# Autodesk Inventor assembly: gantry_frame
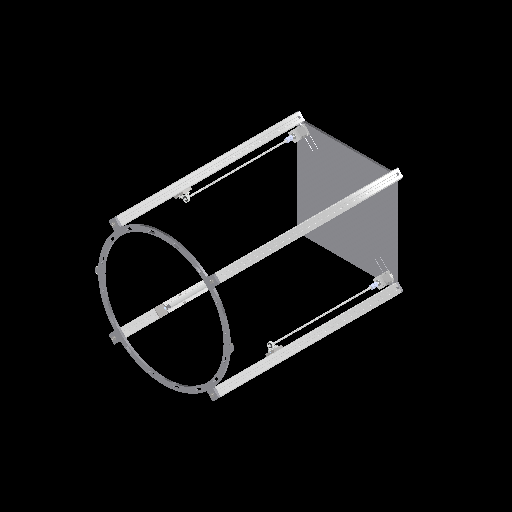
[picture p0: Inventor's stored thumbnail of the model, 512x512]
Saved by Autodesk Inventor 2026.1 (Build 301233000, 233)
## iProperties
Created: 2025-09-18
Part Number: gantry_frame
Document SubType Name: Assembly
Designer: drago
Author: drago
## Documents named in this file (11)
- C:\Users\drago\Desktop\_QIST4500_Multidisciplinary_Team_Project\Proteox MX magnet positioner CAD\magnet_positioner_cad_design\gantry_frame\gantry_frame.iam
- C:\Users\drago\Desktop\_QIST4500_Multidisciplinary_Team_Project\Proteox MX magnet positioner CAD\magnet_positioner_cad_design\gantry_frame\square_bar.ipt
- C:\Users\drago\Desktop\_QIST4500_Multidisciplinary_Team_Project\Proteox MX magnet positioner CAD\magnet_positioner_cad_design\gantry_frame\base_plate.ipt
- C:\Users\drago\Desktop\_QIST4500_Multidisciplinary_Team_Project\Proteox MX magnet positioner CAD\magnet_positioner_cad_design\z_rail\z_rail.iam
- C:\Users\drago\Desktop\_QIST4500_Multidisciplinary_Team_Project\Proteox MX magnet positioner CAD\magnet_positioner_cad_design\gantry_frame\full_ring.iam
- C:\Users\drago\Desktop\_QIST4500_Multidisciplinary_Team_Project\Proteox MX magnet positioner CAD\magnet_positioner_cad_design\z_translator\z_translator.iam
- C:\Users\drago\Documents\Inventor\Content Center Files\R2026\en-US\ISO 7089\ISO 7089 - 8 - 140 HV(1).ipt
- C:\Users\drago\Documents\Inventor\Content Center Files\R2026\en-US\ISO 4762(2)\ISO 4762 - M8 x 30ISO.ipt
- C:\Users\drago\Documents\Inventor\Content Center Files\R2026\en-US\ISO 7089\ISO 7089 - 3 - 140 HV(1).ipt
- C:\Users\drago\Documents\Inventor\Content Center Files\R2026\en-US\ISO 4762(2)\ISO 4762 - M3 x 16ISO.ipt
- C:\Users\drago\Documents\Inventor\Content Center Files\R2026\en-US\ISO 4762(2)\ISO 4762 - M3 x 12ISO.ipt
## Components (42 placed, 10 different names)
1. full_ring:1 [sub-assembly] — Mate:60, Mate:61, Mate:70, Mate:71, Mate:90, Mate:92, Mate:94, Mate:96
2. base_plate:1 — Mate:65, Angle:2, Mate:66, Mate:67, Mate:72, Mate:75, Mate:80, Mate:85, Mate:86, Mate:87, Mate:88, Mate:98, Mate:100, Mate:102, Mate:104, Mate:106, Mate:108, Mate:110, Mate:112, Mate:114, Mate:116, Mate:118, Mate:120
3. z_rail:1 [sub-assembly] — Mate:84, Mate:86, Mate:85
4. z_rail:2 [sub-assembly] — Mate:83, Mate:87, Mate:88
5. z_translator:1 [sub-assembly] — Mate:67, Mate:80, Mate:82, Mate:113, Mate:115, Mate:117, Mate:119
6. z_translator:2 [sub-assembly] — Mate:66, Mate:75, Mate:81, Mate:105, Mate:107, Mate:109, Mate:111
7. ISO 7089 8:1 — Mate:89, Mate:90, Insert:1
8. ISO 4762 M8 x 30:1 — Insert:1
9. ISO 7089 8:2 — Mate:91, Mate:92, Insert:2
10. ISO 4762 M8 x 30:2 — Insert:2
11. ISO 7089 8:3 — Mate:93, Mate:94, Insert:3
12. ISO 4762 M8 x 30:3 — Insert:3
13. ISO 7089 8:4 — Mate:95, Mate:96, Insert:4
14. ISO 4762 M8 x 30:4 — Insert:4
15. ISO 7089 8:5 — Mate:97, Mate:98, Insert:5
16. ISO 4762 M8 x 30:5 — Insert:5
17. ISO 7089 8:6 — Mate:99, Mate:100, Insert:6
18. ISO 4762 M8 x 30:6 — Insert:6
19. ISO 7089 8:7 — Mate:101, Mate:102, Insert:7
20. ISO 4762 M8 x 30:7 — Insert:7
21. ISO 7089 8:8 — Mate:103, Mate:104, Insert:8
22. ISO 4762 M8 x 30:8 — Insert:8
23. ISO 7089 3:1 — Mate:105, Mate:106, Insert:9
24. ISO 4762 M3 x 16:1 — Insert:9
25. ISO 7089 3:2 — Mate:107, Mate:108, Insert:10
26. ISO 4762 M3 x 12:1 — Insert:10
27. ISO 7089 3:3 — Mate:109, Mate:110, Insert:11
28. ISO 4762 M3 x 12:2 — Insert:11
29. ISO 7089 3:4 — Mate:111, Mate:112, Insert:12
30. ISO 4762 M3 x 12:3 — Insert:12
31. ISO 7089 3:5 — Mate:113, Mate:114, Insert:13
32. ISO 4762 M3 x 12:4 — Insert:13
33. ISO 7089 3:6 — Mate:115, Mate:116, Insert:14
34. ISO 4762 M3 x 12:5 — Insert:14
35. ISO 7089 3:7 — Mate:117, Mate:118, Insert:15
36. ISO 4762 M3 x 12:6 — Insert:15
37. ISO 7089 3:8 — Mate:119, Mate:120, Insert:16
38. ISO 4762 M3 x 12:7 — Insert:16
39. square_bar:1 — Mate:70, Mate:71, Angle:3, Mate:72, Mate:83, Mate:91, Mate:99
40. square_bar:2 — Mate:82, Mate:93, Mate:101
41. square_bar:3 — Mate:84, Mate:95, Mate:103
42. square_bar:4 — Mate:81, Mate:89, Mate:97
## Component patterns: (4 elements, first: square_bar:1)
## Relationships (68: Mate 50, Insert 16, Angle 2)
- Mate:60: full_ring:1
- Mate:61: full_ring:1
- Mate:65: base_plate:1
- Angle:2 (45 deg): base_plate:1
- Mate:66: base_plate:1 ↔ z_translator:2
- Mate:67: base_plate:1 ↔ z_translator:1
- Mate:70: full_ring:1 ↔ square_bar:1
- Mate:71: full_ring:1 ↔ square_bar:1
- Angle:3 (45 deg): square_bar:1
- Mate:72: base_plate:1 ↔ square_bar:1
- Mate:75: base_plate:1 ↔ z_translator:2
- Mate:80: base_plate:1 ↔ z_translator:1
- Mate:81: z_translator:2 ↔ square_bar:4
- Mate:82: z_translator:1 ↔ square_bar:2
- Mate:83: z_rail:2 ↔ square_bar:1
- Mate:84: z_rail:1 ↔ square_bar:3
- Mate:86 (-20 mm): base_plate:1 ↔ z_rail:1
- Mate:85: base_plate:1 ↔ z_rail:1
- Mate:87: base_plate:1 ↔ z_rail:2
- Mate:88 (20 mm): base_plate:1 ↔ z_rail:2
- Mate:89: ISO 7089 8:1 ↔ square_bar:4
- Mate:90: full_ring:1 ↔ ISO 7089 8:1
- Insert:1: ISO 7089 8:1 ↔ ISO 4762 M8 x 30:1
- Mate:91: ISO 7089 8:2 ↔ square_bar:1
- Mate:92: full_ring:1 ↔ ISO 7089 8:2
- Insert:2: ISO 7089 8:2 ↔ ISO 4762 M8 x 30:2
- Mate:93: ISO 7089 8:3 ↔ square_bar:2
- Mate:94: full_ring:1 ↔ ISO 7089 8:3
- Insert:3: ISO 7089 8:3 ↔ ISO 4762 M8 x 30:3
- Mate:95: ISO 7089 8:4 ↔ square_bar:3
- Mate:96: full_ring:1 ↔ ISO 7089 8:4
- Insert:4: ISO 7089 8:4 ↔ ISO 4762 M8 x 30:4
- Mate:97: ISO 7089 8:5 ↔ square_bar:4
- Mate:98: base_plate:1 ↔ ISO 7089 8:5
- Insert:5: ISO 7089 8:5 ↔ ISO 4762 M8 x 30:5
- Mate:99: ISO 7089 8:6 ↔ square_bar:1
- Mate:100: base_plate:1 ↔ ISO 7089 8:6
- Insert:6: ISO 7089 8:6 ↔ ISO 4762 M8 x 30:6
- Mate:101: ISO 7089 8:7 ↔ square_bar:2
- Mate:102: base_plate:1 ↔ ISO 7089 8:7
- Insert:7: ISO 7089 8:7 ↔ ISO 4762 M8 x 30:7
- Mate:103: ISO 7089 8:8 ↔ square_bar:3
- Mate:104: base_plate:1 ↔ ISO 7089 8:8
- Insert:8: ISO 7089 8:8 ↔ ISO 4762 M8 x 30:8
- Mate:105: z_translator:2 ↔ ISO 7089 3:1
- Mate:106: base_plate:1 ↔ ISO 7089 3:1
- Insert:9: ISO 7089 3:1 ↔ ISO 4762 M3 x 16:1
- Mate:107: z_translator:2 ↔ ISO 7089 3:2
- Mate:108: base_plate:1 ↔ ISO 7089 3:2
- Insert:10: ISO 7089 3:2 ↔ ISO 4762 M3 x 12:1
- Mate:109: z_translator:2 ↔ ISO 7089 3:3
- Mate:110: base_plate:1 ↔ ISO 7089 3:3
- Insert:11: ISO 7089 3:3 ↔ ISO 4762 M3 x 12:2
- Mate:111: z_translator:2 ↔ ISO 7089 3:4
- Mate:112: base_plate:1 ↔ ISO 7089 3:4
- Insert:12: ISO 7089 3:4 ↔ ISO 4762 M3 x 12:3
- Mate:113: z_translator:1 ↔ ISO 7089 3:5
- Mate:114: base_plate:1 ↔ ISO 7089 3:5
- Insert:13: ISO 7089 3:5 ↔ ISO 4762 M3 x 12:4
- Mate:115: z_translator:1 ↔ ISO 7089 3:6
- Mate:116: base_plate:1 ↔ ISO 7089 3:6
- Insert:14: ISO 7089 3:6 ↔ ISO 4762 M3 x 12:5
- Mate:117: z_translator:1 ↔ ISO 7089 3:7
- Mate:118: base_plate:1 ↔ ISO 7089 3:7
- Insert:15: ISO 7089 3:7 ↔ ISO 4762 M3 x 12:6
- Mate:119: z_translator:1 ↔ ISO 7089 3:8
- Mate:120: base_plate:1 ↔ ISO 7089 3:8
- Insert:16: ISO 7089 3:8 ↔ ISO 4762 M3 x 12:7
